# Autodesk Inventor assembly: Ручной привод
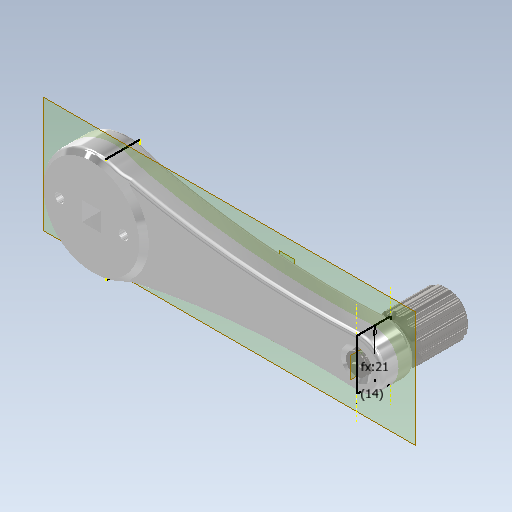
[picture p0: Inventor's stored thumbnail of the model, 512x512]
Saved by Autodesk Inventor 2021 (Build 250183000, 183)
## iProperties
Created: 2020-12-08
Part Number: Ручной привод
Document SubType Name: Assembly
Designer: User
Author: User
## Documents named in this file (5)
- F:\Vise\Модели\Тиски\Ручной привод.iam
- F:\Vise\Модели\Тиски\Ручка привода.ipt
- F:\Vise\Модели\Тиски\Ручной привод\Мастер проектирования\Подшипник1.iam
- F:\Vise\Модели\Тиски\Ручка ручного привода.ipt
- C:\Users\User\Documents\Inventor\Content Center Files\R2020\ru-RU\AS 1427(04)\AS 1427 - M5 x 35(5) I.ipt
## Components (5 placed, 4 different names)
1. Ручка привода:1 — Заподлицо:1, Заподлицо:3, Заподлицо:4, Совмещение:1, Жесткий:2
2. Подшипник:1 [sub-assembly] — Жесткий:2, Жесткий:3
3. Подшипник:2 [sub-assembly] — Заподлицо:2
4. Ручка ручного привода:1 — Заподлицо:1, Заподлицо:2
5. AS 1427 H - метрическая M5 x 35:1 — Жесткий:3
## Relationships (7: Flush 4, WeldJoint 2, Mate 1)
- Заподлицо:1 [Flush]: Ручка привода:1 ↔ Ручка ручного привода:1
- Заподлицо:2 [Flush]: Подшипник:2 ↔ Ручка ручного привода:1
- Заподлицо:3 [Flush]: Ручка привода:1
- Заподлицо:4 [Flush]: Ручка привода:1
- Совмещение:1 [Mate]: Ручка привода:1
- Жесткий:2 [WeldJoint] (0.6 mm): Ручка привода:1 ↔ Подшипник:1
- Жесткий:3 [WeldJoint]: Подшипник:1 ↔ AS 1427 H - метрическая M5 x 35:1
